# Autodesk Inventor assembly: FORMA
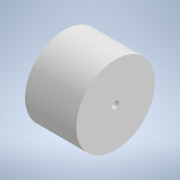
[picture p0: Inventor's stored thumbnail of the model, 180x180]
Saved by Autodesk Inventor 2022 (Build 260153000, 153)
## iProperties
Created: 2023-01-23
Part Number: FORMA
Document SubType Name: Assembly
Designer: Kamil
Author: Kamil
## Documents named in this file (3)
- C:\Users\Kamil\Desktop\FORMA.iam
- C:\Users\Kamil\Desktop\KÓŁKO_STEFAN_NOWE_DO_FORMY.ipt
- C:\Users\Kamil\Documents\Inventor\Forma.ipt
## Components (2 placed, 2 different names)
1. KÓŁKO_STEFAN_NOWE_DO_FORMY:1 — Flush:1
2. Forma:1 — Flush:1
## Relationships (1: Flush 1)
- Flush:1: KÓŁKO_STEFAN_NOWE_DO_FORMY:1 ↔ Forma:1
